# Autodesk Inventor assembly: brazo robot
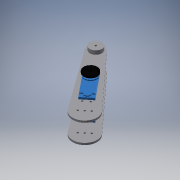
[picture p0: Inventor's stored thumbnail of the model, 180x180]
Saved by Autodesk Inventor 2018 (Build 220112000, 112)
## iProperties
Created: 2020-03-10
Part Number: brazo robot
Material: Genérico
Document SubType Name: Assembly
Designer: sala.ceri
Author: sala.ceri
## Documents named in this file (6)
- C:\Users\david\OneDrive\Documents\robot\ensamble\part3.iam
- C:\Users\david\OneDrive\Documents\robot\piezas\ServoMotor.ipt
- C:\Users\david\OneDrive\Documents\robot\brazo1.ipt
- C:\Users\david\OneDrive\Documents\robot\piezas\BaseServo.ipt
- C:\Users\david\OneDrive\Documents\robot\brazo.ipt
- C:\Users\david\OneDrive\Documents\robot\rosquilla.ipt
## Components (6 placed, 5 different names)
1. brazo1:1 — Coincidencia:28, Coincidencia:29, Coincidencia:30, Coincidencia:32
2. ServoMotor:3 — Coincidencia:28, Coincidencia:29, Coincidencia:39
3. brazo:1
4. rosquilla:1 — Coincidencia:30, Coincidencia:31, Coincidencia:32, Coincidencia:33
5. rosquilla:2 — Coincidencia:31, Coincidencia:33
6. BaseServo:3 — Coincidencia:39
## Relationships (7: Mate 7)
- Coincidencia:28 [Mate]: brazo1:1 ↔ ServoMotor:3
- Coincidencia:29 [Mate]: brazo1:1 ↔ ServoMotor:3
- Coincidencia:30 [Mate]: brazo1:1 ↔ rosquilla:1
- Coincidencia:31 [Mate]: rosquilla:1 ↔ rosquilla:2
- Coincidencia:32 [Mate]: brazo1:1 ↔ rosquilla:1
- Coincidencia:33 [Mate]: rosquilla:1 ↔ rosquilla:2
- Coincidencia:39 [Mate]: ServoMotor:3 ↔ BaseServo:3
